# Autodesk Inventor assembly: 4 overgange
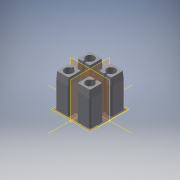
[picture p0: Inventor's stored thumbnail of the model, 180x180]
Saved by Autodesk Inventor 2019 (Build 230136000, 136)
## iProperties
Created: 2019-03-12
Part Number: 4 overgange
Document SubType Name: Assembly
Designer: jonas
Author: jonas
## Documents named in this file (5)
- C:\Users\jonas\Desktop\Teknik\Eksamens projekt\4 overgange.iam
- C:\Users\jonas\Desktop\Teknik\Eksamens projekt\hjul-motor overgang.ipt
- C:\Users\jonas\Desktop\Teknik\Eksamens projekt\hjul-motor overgang_MIR.ipt
- C:\Users\jonas\Desktop\Teknik\Eksamens projekt\hjul-motor overgang_MIR1.ipt
- C:\Users\jonas\Desktop\Teknik\Eksamens projekt\hjul-motor overgang_MIR_MIR.ipt
## Components (4 placed, 4 different names)
1. hjul-motor overgang:3 — Mate:4
2. hjul-motor overgang_MIR:1 — Mate:5
3. hjul-motor overgang_MIR1:1 — Mate:6
4. hjul-motor overgang_MIR_MIR:1 — Mate:7
## Relationships (4: Mate 4)
- Mate:4: hjul-motor overgang:3
- Mate:5: hjul-motor overgang_MIR:1
- Mate:6: hjul-motor overgang_MIR1:1
- Mate:7: hjul-motor overgang_MIR_MIR:1
